# Autodesk Inventor assembly: am14u3LongWithCube
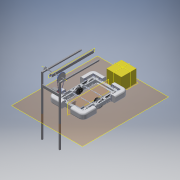
[picture p0: Inventor's stored thumbnail of the model, 180x180]
Saved by Autodesk Inventor 2018.2 (Build 222227000, 227)
## iProperties
Created: 2018-01-10
Part Number: am14u3LongWithCube
Document SubType Name: Assembly
Designer: steele
Author: steele
## Documents named in this file (3)
- D:\snobotics\CAD-Development\robSteele\2018-FRC\am14u3LongWithCube.iam
- D:\snobotics\CAD-Development\robSteele\2018-FRC\AM14U3 Long with Bumper\DB_DriveBaseLong_AM14U3_Bumpers and Battery Tray.iam
- D:\snobotics\CAD-Development\robSteele\2018-FRC\Field Elements\Cube-GE-18124.ipt
## Components (2 placed, 2 different names)
1. DB_DriveBaseLong_AM14U3_Bumpers and Battery Tray:1 [sub-assembly] — Mate:1, Mate:2
2. Cube-GE-18124:1 — Mate:1, Flush:1, Mate:2
## Relationships (3: Mate 2, Flush 1)
- Mate:1: DB_DriveBaseLong_AM14U3_Bumpers and Battery Tray:1 ↔ Cube-GE-18124:1
- Flush:1: Cube-GE-18124:1
- Mate:2 (152.4 mm): DB_DriveBaseLong_AM14U3_Bumpers and Battery Tray:1 ↔ Cube-GE-18124:1
